# Autodesk Inventor assembly: 15x15
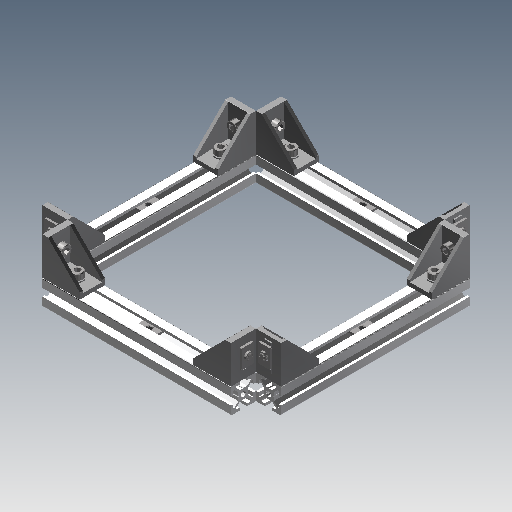
[picture p0: Inventor's stored thumbnail of the model, 512x512]
Saved by Autodesk Inventor 2017 (Build 210142000, 142)
## iProperties
Created: 2016-07-21
Part Number: 15x15
Document SubType Name: Assembly
Designer: Jonathan
Author: Jonathan
## Documents named in this file (4)
- C:\Users\sawaiz\oneDrive\projects\muonTelescope\frame\shapes\15x15.iam
- C:\Users\sawaiz\oneDrive\projects\muonTelescope\frame\extrusions\15 cm extrusion.ipt
- C:\Users\sawaiz\oneDrive\projects\muonTelescope\frame\brackets\angleBracket.iam
- C:\Users\sawaiz\oneDrive\projects\muonTelescope\frame\brackets\m5TNut.ipt
## Components (20 placed, 3 different names)
1. 15 cm extrusion:1 — Mate:9, Mate:16, Flush:14, Flush:21, Flush:27, Mate:17, Mate:18, Symmetry:2, Flush:31, Flush:32, Mate:20, Flush:34, Mate:23, Mate:24
2. 15 cm extrusion:2 — Mate:12, Mate:13, Flush:17, Flush:18, Flush:24, Flush:26, Symmetry:2, Flush:30, Flush:31, Flush:32, Mate:19, Mate:21, Mate:22
3. 15 cm extrusion:3 — Mate:14, Mate:15, Flush:15, Flush:16, Flush:25, Flush:28, Symmetry:1, Symmetry:3, Flush:29, Flush:30, Flush:33, Mate:21
4. 15 cm extrusion:4 — Mate:10, Mate:11, Flush:19, Flush:20, Flush:22, Flush:23, Symmetry:1, Symmetry:3, Flush:29, Flush:33, Mate:19, Mate:20, Mate:22
5. angleBracket:5 [sub-assembly] — Mate:9, Flush:21, Flush:34, Flush:35
6. angleBracket:6 [sub-assembly] — Mate:10, Flush:20, Flush:22
7. angleBracket:7 [sub-assembly] — Mate:11, Flush:19, Flush:23
8. angleBracket:8 [sub-assembly] — Mate:12, Flush:18, Flush:24
9. angleBracket:9 [sub-assembly] — Mate:13, Flush:17, Flush:26
10. angleBracket:10 [sub-assembly] — Mate:14, Flush:16, Flush:25
11. angleBracket:11 [sub-assembly] — Mate:15, Flush:15, Flush:28
12. angleBracket:12 [sub-assembly] — Mate:16, Flush:14, Flush:27
13. m5TNut:1 — Mate:17, Mate:18, Flush:35, Flush:36
14. m5TNut:2 — Mate:23, Mate:24, Flush:36
15. m5TNut:3
16. m5TNut:4
17. m5TNut:5
18. m5TNut:6
19. m5TNut:7
20. m5TNut:8
## Component patterns: (4 elements, first: m5TNut:1 + m5TNut:2)
## Relationships (42: Flush 23, Mate 16, Symmetry 3)
- Mate:9: 15 cm extrusion:1 ↔ angleBracket:5
- Mate:10: 15 cm extrusion:4 ↔ angleBracket:6
- Mate:11: 15 cm extrusion:4 ↔ angleBracket:7
- Mate:12: 15 cm extrusion:2 ↔ angleBracket:8
- Mate:13: 15 cm extrusion:2 ↔ angleBracket:9
- Mate:14: 15 cm extrusion:3 ↔ angleBracket:10
- Mate:15: 15 cm extrusion:3 ↔ angleBracket:11
- Mate:16: 15 cm extrusion:1 ↔ angleBracket:12
- Flush:14: 15 cm extrusion:1 ↔ angleBracket:12
- Flush:15: 15 cm extrusion:3 ↔ angleBracket:11
- Flush:16: 15 cm extrusion:3 ↔ angleBracket:10
- Flush:17: 15 cm extrusion:2 ↔ angleBracket:9
- Flush:18: 15 cm extrusion:2 ↔ angleBracket:8
- Flush:19: 15 cm extrusion:4 ↔ angleBracket:7
- Flush:20: 15 cm extrusion:4 ↔ angleBracket:6
- Flush:21: 15 cm extrusion:1 ↔ angleBracket:5
- Flush:22: 15 cm extrusion:4 ↔ angleBracket:6
- Flush:23: 15 cm extrusion:4 ↔ angleBracket:7
- Flush:24: 15 cm extrusion:2 ↔ angleBracket:8
- Flush:25: 15 cm extrusion:3 ↔ angleBracket:10
- Flush:26: 15 cm extrusion:2 ↔ angleBracket:9
- Flush:27: 15 cm extrusion:1 ↔ angleBracket:12
- Flush:28: 15 cm extrusion:3 ↔ angleBracket:11
- Mate:17: 15 cm extrusion:1 ↔ m5TNut:1
- Mate:18 (1 mm): 15 cm extrusion:1 ↔ m5TNut:1
- Symmetry:1: 15 cm extrusion:3 ↔ 15 cm extrusion:4
- Symmetry:2: 15 cm extrusion:1 ↔ 15 cm extrusion:2
- Symmetry:3: 15 cm extrusion:3 ↔ 15 cm extrusion:4
- Flush:29: 15 cm extrusion:3 ↔ 15 cm extrusion:4
- Flush:30: 15 cm extrusion:2 ↔ 15 cm extrusion:3
- Flush:31: 15 cm extrusion:1 ↔ 15 cm extrusion:2
- Flush:32: 15 cm extrusion:1 ↔ 15 cm extrusion:2
- Flush:33: 15 cm extrusion:3 ↔ 15 cm extrusion:4
- Mate:19: 15 cm extrusion:2 ↔ 15 cm extrusion:4
- Mate:20: 15 cm extrusion:1 ↔ 15 cm extrusion:4
- Mate:21: 15 cm extrusion:2 ↔ 15 cm extrusion:3
- Mate:22: 15 cm extrusion:2 ↔ 15 cm extrusion:4
- Flush:34: 15 cm extrusion:1 ↔ angleBracket:5
- Flush:35 (67.5 mm): angleBracket:5 ↔ m5TNut:1
- Mate:23 (1 mm): 15 cm extrusion:1 ↔ m5TNut:2
- Mate:24: 15 cm extrusion:1 ↔ m5TNut:2
- Flush:36: m5TNut:1 ↔ m5TNut:2
